# Autodesk Inventor assembly: #Spindexer
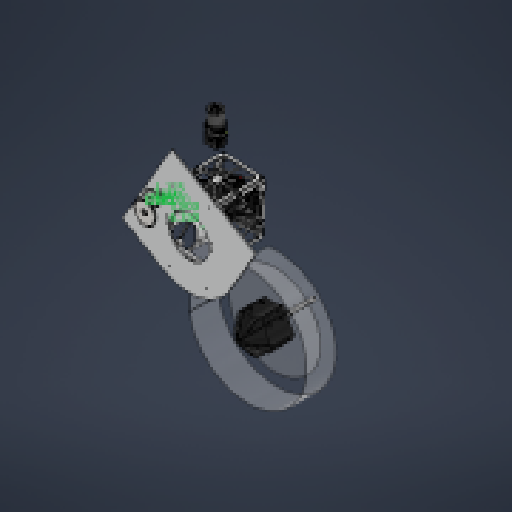
[picture p0: Inventor's stored thumbnail of the model, 512x512]
Saved by Autodesk Inventor 2026 (Build 300175000, 175)
## iProperties
Created: 2026-02-05
Part Number: #Spindexer
Document SubType Name: Assembly
Designer: Owen L
Mass: 5238.72 g
Surface Area: 14057.1 cm^2
Volume: 4457.84 cm^3
Density: 1.17517 g/cm^3
Author: Owen L
## Documents named in this file (44)
- C:\Users\littl\OneDrive\Documents\GitHub\2026-Robot-Mechanical\Spindexer\#Spindexer.iam
- C:\Users\littl\OneDrive\Documents\GitHub\2026-Robot-Mechanical\Spindexer\3DPRINT,HUB.ipt
- C:\Users\littl\OneDrive\Documents\GitHub\2026-Robot-Mechanical\Spindexer\3DPRINT,HUB,CONE.ipt
- C:\Users\littl\OneDrive\Documents\GitHub\2026-Robot-Mechanical\Spindexer\PLATE,WALL.ipt
- C:\Users\littl\OneDrive\Documents\GitHub\2026-Robot-Mechanical\Spindexer\PLATE,BOTTOM.ipt
- C:\Users\littl\OneDrive\Documents\GitHub\2026-Robot-Mechanical\Spindexer\STOCK,HEX,SHAFT,HUB.ipt
- C:\Users\littl\OneDrive\Documents\GitHub\2026-Robot-Mechanical\Spindexer\TEMP,BASE-SKETCH,TANGENT-OUT.ipt
- C:\Users\littl\OneDrive\Documents\GitHub\2026-Robot-Mechanical\Spindexer\PLATE,KICKER,OUTSIDE.ipt
- C:\Users\littl\OneDrive\Documents\GitHub\2026-Robot-Mechanical\Spindexer\3DPRINT,KICKER,RAMP.ipt
- C:\Users\littl\OneDrive\Documents\GitHub\2026-Robot-Mechanical\Spindexer\PLATE,KICKER,INSIDE.ipt
- C:\Users\littl\OneDrive\Documents\GitHub\2026-Robot-Mechanical\Spindexer\STOCK,HEX,SHAFT,KICKER,FRONT.ipt
- C:\Users\littl\OneDrive\Documents\GitHub\2026-Robot-Mechanical\Spindexer\STOCK,HEX,SHAFT,KICKER,BACK.ipt
- C:\Users\littl\OneDrive\Documents\GitHub\2026-Robot-Mechanical\#1_CAD Library\Power Transmission\Bearings\PURCHASED,HEX_BEARING.ipt
- C:\Users\littl\OneDrive\Documents\GitHub\2026-Robot-Mechanical\#1_CAD Library\Power Transmission\VersaPlanetary\GEARBOX,VERSAPLANETARY,SINGLE-STAGE,HEX-SHAFT,0.5IN.ipt
- C:\Users\littl\OneDrive\Documents\GitHub\2026-Robot-Mechanical\#1_CAD Library\Power Transmission\VersaPlanetary\ADAPTER,CIM-NEO,VERSAPLANETARY.ipt
- C:\Users\littl\OneDrive\Documents\GitHub\2026-Robot-Mechanical\#1_CAD Library\Motors\MOTOR,REV,NEO,V1-1.ipt
- C:\Users\littl\OneDrive\Documents\GitHub\2026-Robot-Mechanical\Spindexer\PLATE,NUT-BLOCK,3-LONG.ipt
- C:\Users\littl\OneDrive\Documents\GitHub\2026-Robot-Mechanical\Spindexer\PLATE,NUT-BLOCK,2-LONG.ipt
- C:\Users\littl\OneDrive\Documents\GitHub\2026-Robot-Mechanical\Spindexer\PLATE,NUT-BLOCK,1-LONG.ipt
- C:\Users\littl\OneDrive\Documents\GitHub\2026-Robot-Mechanical\#1_CAD Library\Electronics\CONTROLS,SPARK_MAX.ipt
- C:\Users\littl\OneDrive\Documents\GitHub\2026-Robot-Mechanical\Spindexer\3DPRINT,SPARK_MAX,MOUNT.ipt
- C:\Users\littl\OneDrive\Documents\GitHub\2026-Robot-Mechanical\Spindexer\PLATE,KICKER,BACK.ipt
- C:\Users\littl\OneDrive\Documents\GitHub\2026-Robot-Mechanical\Spindexer\PLATE,NUT-BLOCK,L-SHAPE.ipt
- C:\Users\littl\OneDrive\Documents\GitHub\2026-Robot-Mechanical\Spindexer\3DPRINTED,PULLEY,21T,9mm.ipt
- C:\Users\littl\OneDrive\Documents\GitHub\2026-Robot-Mechanical\#1_CAD Library\Power Transmission\Pulleys\PURCHASED,HTD5mm,24T,PULLEY.ipt
- C:\Users\littl\OneDrive\Documents\GitHub\2026-Robot-Mechanical\Spindexer\STANDIN,BELT,70T,HTD5mm.ipt
- C:\Users\littl\OneDrive\Documents\GitHub\2026-Robot-Mechanical\Spindexer\STANDIN,BELT,100T,HTD5mm.ipt
- C:\Users\littl\OneDrive\Documents\GitHub\2026-Robot-Mechanical\#1_CAD Library\Building Materials\Fasteners\Bolts\PURCHASED,10-32x0.5in,BUTTONHEAD,BOLT.ipt
- C:\Users\littl\OneDrive\Documents\GitHub\2026-Robot-Mechanical\#1_CAD Library\Building Materials\Fasteners\Nuts\PURCHASED,NYLOCK,10-32,NUT.ipt
- C:\Users\littl\OneDrive\Documents\GitHub\2026-Robot-Mechanical\#1_CAD Library\Building Materials\Fasteners\Bolts\PURCHASED,10-32x0.625in,BUTTONHEAD,BOLT.ipt
- C:\Users\littl\OneDrive\Documents\GitHub\2026-Robot-Mechanical\Spindexer\PLATE,NUT-BLOCK,SINGLE-L.ipt
- C:\Users\littl\OneDrive\Documents\GitHub\2026-Robot-Mechanical\Spindexer\PLATE,SHOOTER,MOUNT.ipt
- C:\Users\littl\OneDrive\Documents\GitHub\2026-Robot-Mechanical\Spindexer\#Spindexer\Design Accelerator\PLATE,TURRET,ENCODER,GEAR.ipt
- C:\Users\littl\OneDrive\Documents\GitHub\2026-Robot-Mechanical\Spindexer\#Spindexer\Design Accelerator\PLATE,TURRET,PINNION,GEAR.ipt
- C:\Users\littl\OneDrive\Documents\GitHub\2026-Robot-Mechanical\Spindexer\#Spindexer\Design Accelerator\PLATE,TURRET,MOTOR,MOUNT.ipt
- C:\Users\littl\OneDrive\Documents\GitHub\2026-Robot-Mechanical\#1_CAD Library\Electronics\CONTROLS,ENCODER,HEX_BORE.ipt
- C:\Users\littl\OneDrive\Documents\GitHub\2026-Robot-Mechanical\Spindexer\#Spindexer\Design Accelerator\STOCK,HEX,SHAFT,TURRET,DRIVE.ipt
- C:\Users\littl\OneDrive\Documents\GitHub\2026-Robot-Mechanical\Spindexer\#Spindexer\Design Accelerator\STOCK,HEX,SHAFT,TURRET,ENCODER.ipt
- C:\Users\littl\OneDrive\Documents\GitHub\2026-Robot-Mechanical\Spindexer\#Spindexer\Design Accelerator\3DPRINT,TURRET,HEX,SPACER.ipt
- C:\Users\littl\OneDrive\Documents\GitHub\2026-Robot-Mechanical\Spindexer\MOTOR,NEO,VORTEX,WITH-MAX-PLANETARY.ipt
- C:\Users\littl\OneDrive\Documents\GitHub\2026-Robot-Mechanical\Spindexer\STOCK,CHURRO,HEX,TURRET,MOTOR-MOUNT,SPACER.ipt
- C:\Users\littl\OneDrive\Documents\GitHub\2026-Robot-Mechanical\#1_CAD Library\Building Materials\Fasteners\Bolts\PURCHASED,0.25-20x0.5in,BUTTONHEAD,BOLT.ipt
- C:\Users\littl\OneDrive\Documents\GitHub\2026-Robot-Mechanical\Spindexer\3DRPINT,FRONT-ROLLER,DRIVE-SPACER.ipt
- C:\Users\littl\OneDrive\Documents\GitHub\2026-Robot-Mechanical\Spindexer\CAST,SLAB-OF-FLOP.ipt
## Components (132 placed, 43 different names)
1. 3DPRINT,HUB:1 — Mate:11, Mate:12, Mate:13, Mate:15, Mate:16, Mate:17, Flush:2, Mate:18, Mate:19, Mate:106, Mate:107, Mate:108, Mate:109, Mate:110, Mate:111, Mate:112, Mate:113, Mate:114, Mate:115
2. 3DPRINT,HUB,CONE:1 — Mate:11, Mate:12, Mate:13
3. PLATE,WALL:1 — Mate:32, Flush:7, Flush:8, Mate:42, Mate:43
4. PLATE,BOTTOM:1 — Mate:18, Mate:19, Mate:32, Flush:7
5. STOCK,HEX,SHAFT,HUB:1 — Mate:16, Mate:17, Flush:2
6. TEMP,BASE-SKETCH,TANGENT-OUT:1
7. PLATE,KICKER,OUTSIDE:1 — Mate:22, Mate:23, Mate:24, Mate:25, Flush:3, Flush:4, Flush:8, Insert:1, Insert:4, Mate:34, Mate:35, Mate:42, Insert:9, Insert:10, Insert:13, Flush:12, Mate:43, Insert:23, Insert:24, Insert:34, Insert:35, Insert:39, Insert:40, Insert:41, Insert:42, Insert:43, Insert:44, Insert:45, Insert:46, Insert:47, Insert:48, Insert:49, Insert:50, Insert:79, Insert:80, Insert:81, Insert:82, Mate:59, Insert:83, Mate:62, Insert:87, Insert:93, Insert:94, Insert:98, Insert:99, Insert:100, Mate:65
8. 3DPRINT,KICKER,RAMP:1 — Mate:22, Mate:23, Mate:24
9. PLATE,KICKER,INSIDE:1 — Mate:25, Flush:3, Flush:4, Insert:2, Insert:3, Mate:39, Mate:40, Mate:41, Insert:14, Insert:21, Insert:22, Insert:31, Insert:32, Insert:33, Mate:48, Mate:52, Insert:61, Insert:65, Insert:66, Insert:67, Insert:68, Insert:69, Insert:70, Insert:71, Insert:72, Insert:73, Insert:74, Insert:75, Insert:76, Insert:77, Insert:78, Mate:60, Insert:84, Mate:61, Insert:90, Insert:91, Insert:92, Insert:95, Insert:96, Insert:97
10. STOCK,HEX,SHAFT,KICKER,FRONT:1 — Mate:34, Mate:45, Flush:15
11. STOCK,HEX,SHAFT,KICKER,BACK:1 — Mate:35, Mate:46, Mate:47, Flush:14
12. PURCHASED,HEX_BEARING:1 — Insert:1, Flush:15
13. PURCHASED,HEX_BEARING:2 — Insert:2, Mate:103, Mate:104
14. PURCHASED,HEX_BEARING:3 — Insert:3, Mate:63
15. PURCHASED,HEX_BEARING:4 — Insert:4, Flush:14
16. GEARBOX,VERSAPLANETARY,SINGLE-STAGE,HEX-SHAFT,0.5IN:1 — Mate:36, Mate:37, Mate:38, Mate:39, Mate:40, Mate:41, Mate:53
17. ADAPTER,CIM-NEO,VERSAPLANETARY:1 — Mate:36, Mate:37, Mate:38, Insert:5
18. MOTOR,REV,NEO,V1-1:1 — Insert:5
19. PLATE,NUT-BLOCK,3-LONG:1 — Mate:60, Insert:84
20. PLATE,NUT-BLOCK,3-LONG:2 — Insert:9, Insert:10
21. PLATE,NUT-BLOCK,3-LONG:3 — Mate:59, Insert:83
22. PLATE,NUT-BLOCK,1-LONG:1 — Insert:13, Flush:11, Flush:12
23. PLATE,NUT-BLOCK,1-LONG:2 — Insert:14, Flush:11
24. PLATE,NUT-BLOCK,3-LONG:4 — Insert:91, Insert:92, Mate:66
25. PLATE,NUT-BLOCK,3-LONG:5 — Insert:93, Insert:94, Mate:67
26. CONTROLS,SPARK_MAX:1
27. 3DPRINT,SPARK_MAX,MOUNT:1
28. PLATE,KICKER,BACK:1 — Mate:44, Insert:25, Insert:26, Insert:27, Insert:28, Insert:51, Insert:52, Insert:53, Insert:54, Insert:55, Insert:59, Insert:60, Insert:85, Insert:86, Insert:88, Insert:89
29. PLATE,NUT-BLOCK,2-LONG:2 — Insert:21, Insert:22, Mate:44, Insert:26
30. PLATE,NUT-BLOCK,2-LONG:3 — Insert:23, Insert:24, Insert:25
31. PLATE,NUT-BLOCK,3-LONG:6 — Insert:27, Insert:28
32. PLATE,NUT-BLOCK,3-LONG:8 — Insert:31, Insert:32
33. PLATE,NUT-BLOCK,L-SHAPE:1 — Insert:33
34. PLATE,NUT-BLOCK,L-SHAPE:2 — Insert:34
35. 3DPRINTED,PULLEY,21T,9mm:1 — Mate:46, Mate:55, Mate:58, Mate:64, Flush:16
36. 3DPRINTED,PULLEY,21T,9mm:2 — Mate:45, Mate:54, Flush:16
37. PURCHASED,HEX_BEARING:5 — Mate:52, Mate:53
38. PURCHASED,HTD5mm,24T,PULLEY:1 — Mate:47, Flush:13, Mate:57, Mate:63, Mate:64
39. PURCHASED,HTD5mm,24T,PULLEY:2 — Mate:48, Flush:13, Mate:56
40. STANDIN,BELT,70T,HTD5mm:1 — Mate:56, Mate:57
41. STANDIN,BELT,100T,HTD5mm:1 — Mate:54, Mate:55, Mate:58
42. PURCHASED,10-32x0.5in,BUTTONHEAD,BOLT:1 — Insert:48
43. PURCHASED,NYLOCK,10-32,NUT:1 — Insert:81
44. PURCHASED,10-32x0.625in,BUTTONHEAD,BOLT:1 — Insert:35
45. PURCHASED,10-32x0.625in,BUTTONHEAD,BOLT:5 — Insert:39
46. PURCHASED,10-32x0.625in,BUTTONHEAD,BOLT:6 — Insert:40
47. PURCHASED,10-32x0.625in,BUTTONHEAD,BOLT:7 — Insert:41
48. PURCHASED,10-32x0.625in,BUTTONHEAD,BOLT:8 — Insert:42
49. PURCHASED,10-32x0.625in,BUTTONHEAD,BOLT:9 — Insert:43
50. PURCHASED,10-32x0.625in,BUTTONHEAD,BOLT:10 — Insert:44
51. PURCHASED,10-32x0.625in,BUTTONHEAD,BOLT:11 — Insert:45
52. PURCHASED,10-32x0.625in,BUTTONHEAD,BOLT:12 — Insert:46
53. PURCHASED,10-32x0.625in,BUTTONHEAD,BOLT:13 — Insert:47
54. PURCHASED,10-32x0.625in,BUTTONHEAD,BOLT:14 — Insert:51
55. PURCHASED,10-32x0.625in,BUTTONHEAD,BOLT:15 — Insert:52
56. PURCHASED,10-32x0.625in,BUTTONHEAD,BOLT:16 — Insert:53
57. PURCHASED,10-32x0.625in,BUTTONHEAD,BOLT:17 — Insert:54
58. PURCHASED,10-32x0.625in,BUTTONHEAD,BOLT:18 — Insert:55
59. PURCHASED,10-32x0.5in,BUTTONHEAD,BOLT:2 — Insert:49
60. PURCHASED,10-32x0.5in,BUTTONHEAD,BOLT:3 — Insert:50
61. PURCHASED,10-32x0.625in,BUTTONHEAD,BOLT:19 — Insert:59
62. PURCHASED,10-32x0.625in,BUTTONHEAD,BOLT:20 — Insert:89
63. PURCHASED,10-32x0.625in,BUTTONHEAD,BOLT:21 — Insert:87
64. PURCHASED,10-32x0.625in,BUTTONHEAD,BOLT:22 — Insert:60
65. PURCHASED,10-32x0.625in,BUTTONHEAD,BOLT:23 — Insert:88
66. PURCHASED,10-32x0.625in,BUTTONHEAD,BOLT:24 — Insert:61
67. PURCHASED,10-32x0.625in,BUTTONHEAD,BOLT:28 — Insert:65
68. PURCHASED,10-32x0.625in,BUTTONHEAD,BOLT:29 — Insert:66
69. PURCHASED,10-32x0.625in,BUTTONHEAD,BOLT:30 — Insert:67
70. PURCHASED,10-32x0.625in,BUTTONHEAD,BOLT:31 — Insert:68
71. PURCHASED,10-32x0.625in,BUTTONHEAD,BOLT:32 — Insert:69
72. PURCHASED,10-32x0.625in,BUTTONHEAD,BOLT:33 — Insert:70
73. PURCHASED,10-32x0.625in,BUTTONHEAD,BOLT:34 — Insert:73
74. PURCHASED,10-32x0.625in,BUTTONHEAD,BOLT:35 — Insert:72
75. PURCHASED,10-32x0.625in,BUTTONHEAD,BOLT:36 — Insert:71
76. PURCHASED,10-32x0.5in,BUTTONHEAD,BOLT:4 — Insert:74
77. PURCHASED,10-32x0.5in,BUTTONHEAD,BOLT:5 — Insert:76
78. PURCHASED,10-32x0.5in,BUTTONHEAD,BOLT:6 — Insert:75
79. PURCHASED,10-32x0.5in,BUTTONHEAD,BOLT:7 — Insert:77
80. PURCHASED,10-32x0.5in,BUTTONHEAD,BOLT:8 — Insert:78
81. PURCHASED,10-32x0.5in,BUTTONHEAD,BOLT:9 — Insert:79
82. PURCHASED,10-32x0.5in,BUTTONHEAD,BOLT:10 — Insert:80
83. PURCHASED,NYLOCK,10-32,NUT:2 — Insert:82
84. PLATE,NUT-BLOCK,SINGLE-L:1 — Insert:85, Mate:61
85. PLATE,NUT-BLOCK,SINGLE-L:2 — Insert:86, Mate:62
86. PURCHASED,10-32x0.625in,BUTTONHEAD,BOLT:37 — Insert:90
87. PURCHASED,10-32x0.625in,BUTTONHEAD,BOLT:38 — Insert:95
88. PURCHASED,10-32x0.625in,BUTTONHEAD,BOLT:39 — Insert:96
89. PURCHASED,10-32x0.625in,BUTTONHEAD,BOLT:40 — Insert:97
90. PURCHASED,10-32x0.625in,BUTTONHEAD,BOLT:41 — Insert:98
91. PURCHASED,10-32x0.625in,BUTTONHEAD,BOLT:42 — Insert:99
92. PURCHASED,10-32x0.625in,BUTTONHEAD,BOLT:43 — Insert:100
93. PLATE,SHOOTER,MOUNT:1 — Mate:65, Mate:66, Mate:67, Insert:101, Insert:102, Mate:82, Mate:85, Insert:118, Insert:119, Mate:95, Mate:97, Mate:98, Mate:99, Mate:100, Insert:122, Insert:123, Insert:124, Insert:125, Insert:126, Insert:128, Insert:129, Insert:130, Mate:105, Insert:136, Insert:137
94. PLATE,TURRET,ENCODER,GEAR:1 — Mate:85, Flush:20, Mate:89, Mate:102
95. PLATE,TURRET,PINNION,GEAR:1 — Mate:86, Flush:18, Mate:88
96. PURCHASED,HEX_BEARING:6 — Insert:101, Mate:83, Mate:86, Mate:93
97. PURCHASED,HEX_BEARING:7 — Insert:102, Mate:94, Mate:96
98. PLATE,TURRET,MOTOR,MOUNT:1 — Mate:98, Mate:99, Insert:120, Mate:100, Insert:121, Mate:101, Insert:127, Insert:131, Insert:132, Insert:133
99. CONTROLS,ENCODER,HEX_BORE:1 — Mate:95, Mate:96, Mate:97, Insert:135, Insert:134
100. CONTROLS,ENCODER,HEX_BORE:2 — Mate:82, Mate:83, Mate:87, Insert:112, Insert:113
101. STOCK,HEX,SHAFT,TURRET,DRIVE:1 — Flush:20, Mate:89, Mate:91
102. STOCK,HEX,SHAFT,TURRET,ENCODER:1 — Flush:18, Mate:87, Mate:88, Mate:92, Flush:21
103. 3DPRINT,TURRET,HEX,SPACER:1 — Mate:91, Mate:94, Mate:102
104. 3DPRINT,TURRET,HEX,SPACER:2 — Mate:92, Mate:93
105. PURCHASED,10-32x0.625in,BUTTONHEAD,BOLT:44 — Insert:112, Mate:105
106. PURCHASED,10-32x0.625in,BUTTONHEAD,BOLT:45 — Insert:113
107. PURCHASED,NYLOCK,10-32,NUT:5 — Insert:118
108. PURCHASED,NYLOCK,10-32,NUT:6 — Insert:119
109. MOTOR,NEO,VORTEX,WITH-MAX-PLANETARY:1 — Insert:121, Mate:101
110. PURCHASED,HEX_BEARING:9 — Insert:120, Flush:21
111. STOCK,CHURRO,HEX,TURRET,MOTOR-MOUNT,SPACER:1 — Insert:122
112. STOCK,CHURRO,HEX,TURRET,MOTOR-MOUNT,SPACER:2 — Insert:123
113. STOCK,CHURRO,HEX,TURRET,MOTOR-MOUNT,SPACER:3 — Insert:124
114. STOCK,CHURRO,HEX,TURRET,MOTOR-MOUNT,SPACER:4 — Insert:125
115. PURCHASED,0.25-20x0.5in,BUTTONHEAD,BOLT:1 — Insert:132
116. PURCHASED,0.25-20x0.5in,BUTTONHEAD,BOLT:2 — Insert:133
117. PURCHASED,0.25-20x0.5in,BUTTONHEAD,BOLT:3 — Insert:131
118. PURCHASED,0.25-20x0.5in,BUTTONHEAD,BOLT:4 — Insert:130
119. PURCHASED,0.25-20x0.5in,BUTTONHEAD,BOLT:5 — Insert:129
120. PURCHASED,0.25-20x0.5in,BUTTONHEAD,BOLT:6 — Insert:128
121. PURCHASED,0.25-20x0.5in,BUTTONHEAD,BOLT:7 — Insert:127
122. PURCHASED,0.25-20x0.5in,BUTTONHEAD,BOLT:8 — Insert:126
123. 3DRPINT,FRONT-ROLLER,DRIVE-SPACER:1 — Mate:103, Mate:104
124. PURCHASED,10-32x0.625in,BUTTONHEAD,BOLT:46 — Insert:134
125. PURCHASED,10-32x0.625in,BUTTONHEAD,BOLT:47 — Insert:135
126. PURCHASED,NYLOCK,10-32,NUT:7 — Insert:136
127. PURCHASED,NYLOCK,10-32,NUT:8 — Insert:137
128. CAST,SLAB-OF-FLOP:1 — Mate:106, Mate:107
129. CAST,SLAB-OF-FLOP:2 — Mate:108, Mate:109
130. CAST,SLAB-OF-FLOP:3 — Mate:110, Mate:111
131. CAST,SLAB-OF-FLOP:4 — Mate:112, Mate:113
132. CAST,SLAB-OF-FLOP:5 — Mate:114, Mate:115
## Relationships (192: Insert 102, Mate 76, Flush 14)
- Mate:11: 3DPRINT,HUB:1 ↔ 3DPRINT,HUB,CONE:1
- Mate:12: 3DPRINT,HUB:1 ↔ 3DPRINT,HUB,CONE:1
- Mate:13: 3DPRINT,HUB:1 ↔ 3DPRINT,HUB,CONE:1
- Mate:15: 3DPRINT,HUB:1
- Mate:16: 3DPRINT,HUB:1 ↔ STOCK,HEX,SHAFT,HUB:1
- Mate:17: 3DPRINT,HUB:1 ↔ STOCK,HEX,SHAFT,HUB:1
- Flush:2 (-12.7 mm): 3DPRINT,HUB:1 ↔ STOCK,HEX,SHAFT,HUB:1
- Mate:18: 3DPRINT,HUB:1 ↔ PLATE,BOTTOM:1
- Mate:19: 3DPRINT,HUB:1 ↔ PLATE,BOTTOM:1
- Mate:22: PLATE,KICKER,OUTSIDE:1 ↔ 3DPRINT,KICKER,RAMP:1
- Mate:23: PLATE,KICKER,OUTSIDE:1 ↔ 3DPRINT,KICKER,RAMP:1
- Mate:24: PLATE,KICKER,OUTSIDE:1 ↔ 3DPRINT,KICKER,RAMP:1
- Mate:25 (158.75 mm): PLATE,KICKER,OUTSIDE:1 ↔ PLATE,KICKER,INSIDE:1
- Flush:3: PLATE,KICKER,OUTSIDE:1 ↔ PLATE,KICKER,INSIDE:1
- Flush:4: PLATE,KICKER,OUTSIDE:1 ↔ PLATE,KICKER,INSIDE:1
- Mate:32: PLATE,WALL:1 ↔ PLATE,BOTTOM:1
- Flush:7 (-6.35 mm): PLATE,WALL:1 ↔ PLATE,BOTTOM:1
- Flush:8: PLATE,WALL:1 ↔ PLATE,KICKER,OUTSIDE:1
- Insert:1: PLATE,KICKER,OUTSIDE:1 ↔ PURCHASED,HEX_BEARING:1
- Insert:2: PLATE,KICKER,INSIDE:1 ↔ PURCHASED,HEX_BEARING:2
- Insert:3: PLATE,KICKER,INSIDE:1 ↔ PURCHASED,HEX_BEARING:3
- Insert:4: PLATE,KICKER,OUTSIDE:1 ↔ PURCHASED,HEX_BEARING:4
- Mate:34: PLATE,KICKER,OUTSIDE:1 ↔ STOCK,HEX,SHAFT,KICKER,FRONT:1
- Mate:35: PLATE,KICKER,OUTSIDE:1 ↔ STOCK,HEX,SHAFT,KICKER,BACK:1
- Mate:36: GEARBOX,VERSAPLANETARY,SINGLE-STAGE,HEX-SHAFT,0.5IN:1 ↔ ADAPTER,CIM-NEO,VERSAPLANETARY:1
- Mate:37: GEARBOX,VERSAPLANETARY,SINGLE-STAGE,HEX-SHAFT,0.5IN:1 ↔ ADAPTER,CIM-NEO,VERSAPLANETARY:1
- Mate:38: GEARBOX,VERSAPLANETARY,SINGLE-STAGE,HEX-SHAFT,0.5IN:1 ↔ ADAPTER,CIM-NEO,VERSAPLANETARY:1
- Insert:5: ADAPTER,CIM-NEO,VERSAPLANETARY:1 ↔ MOTOR,REV,NEO,V1-1:1
- Mate:39: PLATE,KICKER,INSIDE:1 ↔ GEARBOX,VERSAPLANETARY,SINGLE-STAGE,HEX-SHAFT,0.5IN:1
- Mate:40: PLATE,KICKER,INSIDE:1 ↔ GEARBOX,VERSAPLANETARY,SINGLE-STAGE,HEX-SHAFT,0.5IN:1
- Mate:41: PLATE,KICKER,INSIDE:1 ↔ GEARBOX,VERSAPLANETARY,SINGLE-STAGE,HEX-SHAFT,0.5IN:1
- Mate:42: PLATE,WALL:1 ↔ PLATE,KICKER,OUTSIDE:1
- Insert:9: PLATE,KICKER,OUTSIDE:1 ↔ PLATE,NUT-BLOCK,3-LONG:2
- Insert:10: PLATE,KICKER,OUTSIDE:1 ↔ PLATE,NUT-BLOCK,3-LONG:2
- Insert:13: PLATE,KICKER,OUTSIDE:1 ↔ PLATE,NUT-BLOCK,1-LONG:1
- Insert:14: PLATE,KICKER,INSIDE:1 ↔ PLATE,NUT-BLOCK,1-LONG:2
- Flush:11: PLATE,NUT-BLOCK,1-LONG:1 ↔ PLATE,NUT-BLOCK,1-LONG:2
- Flush:12: PLATE,KICKER,OUTSIDE:1 ↔ PLATE,NUT-BLOCK,1-LONG:1
- Mate:43 (-25.4 mm): PLATE,WALL:1 ↔ PLATE,KICKER,OUTSIDE:1
- Insert:21: PLATE,KICKER,INSIDE:1 ↔ PLATE,NUT-BLOCK,2-LONG:2
- Insert:22: PLATE,KICKER,INSIDE:1 ↔ PLATE,NUT-BLOCK,2-LONG:2
- Insert:23: PLATE,KICKER,OUTSIDE:1 ↔ PLATE,NUT-BLOCK,2-LONG:3
- Insert:24: PLATE,KICKER,OUTSIDE:1 ↔ PLATE,NUT-BLOCK,2-LONG:3
- Mate:44: PLATE,KICKER,BACK:1 ↔ PLATE,NUT-BLOCK,2-LONG:2
- Insert:25: PLATE,KICKER,BACK:1 ↔ PLATE,NUT-BLOCK,2-LONG:3
- Insert:26: PLATE,KICKER,BACK:1 ↔ PLATE,NUT-BLOCK,2-LONG:2
- Insert:27: PLATE,KICKER,BACK:1 ↔ PLATE,NUT-BLOCK,3-LONG:6
- Insert:28: PLATE,KICKER,BACK:1 ↔ PLATE,NUT-BLOCK,3-LONG:6
- Insert:31: PLATE,KICKER,INSIDE:1 ↔ PLATE,NUT-BLOCK,3-LONG:8
- Insert:32: PLATE,KICKER,INSIDE:1 ↔ PLATE,NUT-BLOCK,3-LONG:8
- Insert:33: PLATE,KICKER,INSIDE:1 ↔ PLATE,NUT-BLOCK,L-SHAPE:1
- Insert:34: PLATE,KICKER,OUTSIDE:1 ↔ PLATE,NUT-BLOCK,L-SHAPE:2
- Mate:45: STOCK,HEX,SHAFT,KICKER,FRONT:1 ↔ 3DPRINTED,PULLEY,21T,9mm:2
- Mate:46: STOCK,HEX,SHAFT,KICKER,BACK:1 ↔ 3DPRINTED,PULLEY,21T,9mm:1
- Mate:47: STOCK,HEX,SHAFT,KICKER,BACK:1 ↔ PURCHASED,HTD5mm,24T,PULLEY:1
- Mate:48: PLATE,KICKER,INSIDE:1 ↔ PURCHASED,HTD5mm,24T,PULLEY:2
- Flush:13: PURCHASED,HTD5mm,24T,PULLEY:1 ↔ PURCHASED,HTD5mm,24T,PULLEY:2
- Flush:14: STOCK,HEX,SHAFT,KICKER,BACK:1 ↔ PURCHASED,HEX_BEARING:4
- Flush:15: STOCK,HEX,SHAFT,KICKER,FRONT:1 ↔ PURCHASED,HEX_BEARING:1
- Mate:52: PLATE,KICKER,INSIDE:1 ↔ PURCHASED,HEX_BEARING:5
- Mate:53: GEARBOX,VERSAPLANETARY,SINGLE-STAGE,HEX-SHAFT,0.5IN:1 ↔ PURCHASED,HEX_BEARING:5
- Mate:54: 3DPRINTED,PULLEY,21T,9mm:2 ↔ STANDIN,BELT,100T,HTD5mm:1
- Mate:55: 3DPRINTED,PULLEY,21T,9mm:1 ↔ STANDIN,BELT,100T,HTD5mm:1
- Mate:56: PURCHASED,HTD5mm,24T,PULLEY:2 ↔ STANDIN,BELT,70T,HTD5mm:1
- Mate:57: PURCHASED,HTD5mm,24T,PULLEY:1 ↔ STANDIN,BELT,70T,HTD5mm:1
- Mate:58: 3DPRINTED,PULLEY,21T,9mm:1 ↔ STANDIN,BELT,100T,HTD5mm:1
- Insert:35: PLATE,KICKER,OUTSIDE:1 ↔ PURCHASED,10-32x0.625in,BUTTONHEAD,BOLT:1
- Insert:39: PLATE,KICKER,OUTSIDE:1 ↔ PURCHASED,10-32x0.625in,BUTTONHEAD,BOLT:5
- Insert:40: PLATE,KICKER,OUTSIDE:1 ↔ PURCHASED,10-32x0.625in,BUTTONHEAD,BOLT:6
- Insert:41: PLATE,KICKER,OUTSIDE:1 ↔ PURCHASED,10-32x0.625in,BUTTONHEAD,BOLT:7
- Insert:42: PLATE,KICKER,OUTSIDE:1 ↔ PURCHASED,10-32x0.625in,BUTTONHEAD,BOLT:8
- Insert:43: PLATE,KICKER,OUTSIDE:1 ↔ PURCHASED,10-32x0.625in,BUTTONHEAD,BOLT:9
- Insert:44: PLATE,KICKER,OUTSIDE:1 ↔ PURCHASED,10-32x0.625in,BUTTONHEAD,BOLT:10
- Insert:45: PLATE,KICKER,OUTSIDE:1 ↔ PURCHASED,10-32x0.625in,BUTTONHEAD,BOLT:11
- Insert:46: PLATE,KICKER,OUTSIDE:1 ↔ PURCHASED,10-32x0.625in,BUTTONHEAD,BOLT:12
- Insert:47: PLATE,KICKER,OUTSIDE:1 ↔ PURCHASED,10-32x0.625in,BUTTONHEAD,BOLT:13
- Insert:48: PLATE,KICKER,OUTSIDE:1 ↔ PURCHASED,10-32x0.5in,BUTTONHEAD,BOLT:1
- Insert:49: PLATE,KICKER,OUTSIDE:1 ↔ PURCHASED,10-32x0.5in,BUTTONHEAD,BOLT:2
- Insert:50: PLATE,KICKER,OUTSIDE:1 ↔ PURCHASED,10-32x0.5in,BUTTONHEAD,BOLT:3
- Insert:51: PLATE,KICKER,BACK:1 ↔ PURCHASED,10-32x0.625in,BUTTONHEAD,BOLT:14
- Insert:52: PLATE,KICKER,BACK:1 ↔ PURCHASED,10-32x0.625in,BUTTONHEAD,BOLT:15
- Insert:53: PLATE,KICKER,BACK:1 ↔ PURCHASED,10-32x0.625in,BUTTONHEAD,BOLT:16
- Insert:54: PLATE,KICKER,BACK:1 ↔ PURCHASED,10-32x0.625in,BUTTONHEAD,BOLT:17
- Insert:55: PLATE,KICKER,BACK:1 ↔ PURCHASED,10-32x0.625in,BUTTONHEAD,BOLT:18
- Insert:59: PLATE,KICKER,BACK:1 ↔ PURCHASED,10-32x0.625in,BUTTONHEAD,BOLT:19
- Insert:60: PLATE,KICKER,BACK:1 ↔ PURCHASED,10-32x0.625in,BUTTONHEAD,BOLT:22
- Insert:61: PLATE,KICKER,INSIDE:1 ↔ PURCHASED,10-32x0.625in,BUTTONHEAD,BOLT:24
- Insert:65: PLATE,KICKER,INSIDE:1 ↔ PURCHASED,10-32x0.625in,BUTTONHEAD,BOLT:28
- Insert:66: PLATE,KICKER,INSIDE:1 ↔ PURCHASED,10-32x0.625in,BUTTONHEAD,BOLT:29
- Insert:67: PLATE,KICKER,INSIDE:1 ↔ PURCHASED,10-32x0.625in,BUTTONHEAD,BOLT:30
- Insert:68: PLATE,KICKER,INSIDE:1 ↔ PURCHASED,10-32x0.625in,BUTTONHEAD,BOLT:31
- Insert:69: PLATE,KICKER,INSIDE:1 ↔ PURCHASED,10-32x0.625in,BUTTONHEAD,BOLT:32
- Insert:70: PLATE,KICKER,INSIDE:1 ↔ PURCHASED,10-32x0.625in,BUTTONHEAD,BOLT:33
- Insert:71: PLATE,KICKER,INSIDE:1 ↔ PURCHASED,10-32x0.625in,BUTTONHEAD,BOLT:36
- Insert:72: PLATE,KICKER,INSIDE:1 ↔ PURCHASED,10-32x0.625in,BUTTONHEAD,BOLT:35
- Insert:73: PLATE,KICKER,INSIDE:1 ↔ PURCHASED,10-32x0.625in,BUTTONHEAD,BOLT:34
- Insert:74: PLATE,KICKER,INSIDE:1 ↔ PURCHASED,10-32x0.5in,BUTTONHEAD,BOLT:4
- Insert:75: PLATE,KICKER,INSIDE:1 ↔ PURCHASED,10-32x0.5in,BUTTONHEAD,BOLT:6
- Insert:76: PLATE,KICKER,INSIDE:1 ↔ PURCHASED,10-32x0.5in,BUTTONHEAD,BOLT:5
- Insert:77: PLATE,KICKER,INSIDE:1 ↔ PURCHASED,10-32x0.5in,BUTTONHEAD,BOLT:7
- Insert:78: PLATE,KICKER,INSIDE:1 ↔ PURCHASED,10-32x0.5in,BUTTONHEAD,BOLT:8
- Insert:79: PLATE,KICKER,OUTSIDE:1 ↔ PURCHASED,10-32x0.5in,BUTTONHEAD,BOLT:9
- Insert:80: PLATE,KICKER,OUTSIDE:1 ↔ PURCHASED,10-32x0.5in,BUTTONHEAD,BOLT:10
- Insert:81: PLATE,KICKER,OUTSIDE:1 ↔ PURCHASED,NYLOCK,10-32,NUT:1
- Insert:82: PLATE,KICKER,OUTSIDE:1 ↔ PURCHASED,NYLOCK,10-32,NUT:2
- Mate:59: PLATE,KICKER,OUTSIDE:1 ↔ PLATE,NUT-BLOCK,3-LONG:3
- Insert:83: PLATE,KICKER,OUTSIDE:1 ↔ PLATE,NUT-BLOCK,3-LONG:3
- Mate:60: PLATE,KICKER,INSIDE:1 ↔ PLATE,NUT-BLOCK,3-LONG:1
- Insert:84: PLATE,KICKER,INSIDE:1 ↔ PLATE,NUT-BLOCK,3-LONG:1
- Insert:85: PLATE,KICKER,BACK:1 ↔ PLATE,NUT-BLOCK,SINGLE-L:1
- Mate:61: PLATE,KICKER,INSIDE:1 ↔ PLATE,NUT-BLOCK,SINGLE-L:1
- Insert:86: PLATE,KICKER,BACK:1 ↔ PLATE,NUT-BLOCK,SINGLE-L:2
- Mate:62: PLATE,KICKER,OUTSIDE:1 ↔ PLATE,NUT-BLOCK,SINGLE-L:2
- Insert:87: PLATE,KICKER,OUTSIDE:1 ↔ PURCHASED,10-32x0.625in,BUTTONHEAD,BOLT:21
- Insert:88: PLATE,KICKER,BACK:1 ↔ PURCHASED,10-32x0.625in,BUTTONHEAD,BOLT:23
- Insert:89: PLATE,KICKER,BACK:1 ↔ PURCHASED,10-32x0.625in,BUTTONHEAD,BOLT:20
- Insert:90: PLATE,KICKER,INSIDE:1 ↔ PURCHASED,10-32x0.625in,BUTTONHEAD,BOLT:37
- Mate:63: PURCHASED,HEX_BEARING:3 ↔ PURCHASED,HTD5mm,24T,PULLEY:1
- Mate:64: 3DPRINTED,PULLEY,21T,9mm:1 ↔ PURCHASED,HTD5mm,24T,PULLEY:1
- Flush:16: 3DPRINTED,PULLEY,21T,9mm:1 ↔ 3DPRINTED,PULLEY,21T,9mm:2
- Insert:91: PLATE,KICKER,INSIDE:1 ↔ PLATE,NUT-BLOCK,3-LONG:4
- Insert:92: PLATE,KICKER,INSIDE:1 ↔ PLATE,NUT-BLOCK,3-LONG:4
- Insert:93: PLATE,KICKER,OUTSIDE:1 ↔ PLATE,NUT-BLOCK,3-LONG:5
- Insert:94: PLATE,KICKER,OUTSIDE:1 ↔ PLATE,NUT-BLOCK,3-LONG:5
- Insert:95: PLATE,KICKER,INSIDE:1 ↔ PURCHASED,10-32x0.625in,BUTTONHEAD,BOLT:38
- Insert:96: PLATE,KICKER,INSIDE:1 ↔ PURCHASED,10-32x0.625in,BUTTONHEAD,BOLT:39
- Insert:97: PLATE,KICKER,INSIDE:1 ↔ PURCHASED,10-32x0.625in,BUTTONHEAD,BOLT:40
- Insert:98: PLATE,KICKER,OUTSIDE:1 ↔ PURCHASED,10-32x0.625in,BUTTONHEAD,BOLT:41
- Insert:99: PLATE,KICKER,OUTSIDE:1 ↔ PURCHASED,10-32x0.625in,BUTTONHEAD,BOLT:42
- Insert:100: PLATE,KICKER,OUTSIDE:1 ↔ PURCHASED,10-32x0.625in,BUTTONHEAD,BOLT:43
- Mate:65: PLATE,KICKER,OUTSIDE:1 ↔ PLATE,SHOOTER,MOUNT:1
- Mate:66: PLATE,NUT-BLOCK,3-LONG:4 ↔ PLATE,SHOOTER,MOUNT:1
- Mate:67: PLATE,NUT-BLOCK,3-LONG:5 ↔ PLATE,SHOOTER,MOUNT:1
- Insert:101: PLATE,SHOOTER,MOUNT:1 ↔ PURCHASED,HEX_BEARING:6
- Insert:102: PLATE,SHOOTER,MOUNT:1 ↔ PURCHASED,HEX_BEARING:7
- Mate:82: PLATE,SHOOTER,MOUNT:1 ↔ CONTROLS,ENCODER,HEX_BORE:2
- Mate:83: PURCHASED,HEX_BEARING:6 ↔ CONTROLS,ENCODER,HEX_BORE:2
- Mate:85: PLATE,SHOOTER,MOUNT:1 ↔ PLATE,TURRET,ENCODER,GEAR:1
- Mate:86: PLATE,TURRET,PINNION,GEAR:1 ↔ PURCHASED,HEX_BEARING:6
- Flush:18: PLATE,TURRET,PINNION,GEAR:1 ↔ STOCK,HEX,SHAFT,TURRET,ENCODER:1
- Mate:87: CONTROLS,ENCODER,HEX_BORE:2 ↔ STOCK,HEX,SHAFT,TURRET,ENCODER:1
- Mate:88: PLATE,TURRET,PINNION,GEAR:1 ↔ STOCK,HEX,SHAFT,TURRET,ENCODER:1
- Flush:20: PLATE,TURRET,ENCODER,GEAR:1 ↔ STOCK,HEX,SHAFT,TURRET,DRIVE:1
- Mate:89: PLATE,TURRET,ENCODER,GEAR:1 ↔ STOCK,HEX,SHAFT,TURRET,DRIVE:1
- Mate:91: STOCK,HEX,SHAFT,TURRET,DRIVE:1 ↔ 3DPRINT,TURRET,HEX,SPACER:1
- Mate:92: STOCK,HEX,SHAFT,TURRET,ENCODER:1 ↔ 3DPRINT,TURRET,HEX,SPACER:2
- Mate:93: PURCHASED,HEX_BEARING:6 ↔ 3DPRINT,TURRET,HEX,SPACER:2
- Mate:94: PURCHASED,HEX_BEARING:7 ↔ 3DPRINT,TURRET,HEX,SPACER:1
- Insert:112: CONTROLS,ENCODER,HEX_BORE:2 ↔ PURCHASED,10-32x0.625in,BUTTONHEAD,BOLT:44
- Insert:113: CONTROLS,ENCODER,HEX_BORE:2 ↔ PURCHASED,10-32x0.625in,BUTTONHEAD,BOLT:45
- Insert:118: PLATE,SHOOTER,MOUNT:1 ↔ PURCHASED,NYLOCK,10-32,NUT:5
- Insert:119: PLATE,SHOOTER,MOUNT:1 ↔ PURCHASED,NYLOCK,10-32,NUT:6
- Mate:95: PLATE,SHOOTER,MOUNT:1 ↔ CONTROLS,ENCODER,HEX_BORE:1
- Mate:96: PURCHASED,HEX_BEARING:7 ↔ CONTROLS,ENCODER,HEX_BORE:1
- Mate:97: PLATE,SHOOTER,MOUNT:1 ↔ CONTROLS,ENCODER,HEX_BORE:1
- Mate:98: PLATE,SHOOTER,MOUNT:1 ↔ PLATE,TURRET,MOTOR,MOUNT:1
- Mate:99: PLATE,SHOOTER,MOUNT:1 ↔ PLATE,TURRET,MOTOR,MOUNT:1
- Insert:120: PLATE,TURRET,MOTOR,MOUNT:1 ↔ PURCHASED,HEX_BEARING:9
- Mate:100 (17.78 mm): PLATE,SHOOTER,MOUNT:1 ↔ PLATE,TURRET,MOTOR,MOUNT:1
- Insert:121: PLATE,TURRET,MOTOR,MOUNT:1 ↔ MOTOR,NEO,VORTEX,WITH-MAX-PLANETARY:1
- Mate:101: PLATE,TURRET,MOTOR,MOUNT:1 ↔ MOTOR,NEO,VORTEX,WITH-MAX-PLANETARY:1
- Flush:21: STOCK,HEX,SHAFT,TURRET,ENCODER:1 ↔ PURCHASED,HEX_BEARING:9
- Mate:102: PLATE,TURRET,ENCODER,GEAR:1 ↔ 3DPRINT,TURRET,HEX,SPACER:1
- Insert:122: PLATE,SHOOTER,MOUNT:1 ↔ STOCK,CHURRO,HEX,TURRET,MOTOR-MOUNT,SPACER:1
- Insert:123: PLATE,SHOOTER,MOUNT:1 ↔ STOCK,CHURRO,HEX,TURRET,MOTOR-MOUNT,SPACER:2
- Insert:124: PLATE,SHOOTER,MOUNT:1 ↔ STOCK,CHURRO,HEX,TURRET,MOTOR-MOUNT,SPACER:3
- Insert:125: PLATE,SHOOTER,MOUNT:1 ↔ STOCK,CHURRO,HEX,TURRET,MOTOR-MOUNT,SPACER:4
- Insert:126: PLATE,SHOOTER,MOUNT:1 ↔ PURCHASED,0.25-20x0.5in,BUTTONHEAD,BOLT:8
- Insert:127: PLATE,TURRET,MOTOR,MOUNT:1 ↔ PURCHASED,0.25-20x0.5in,BUTTONHEAD,BOLT:7
- Insert:128: PLATE,SHOOTER,MOUNT:1 ↔ PURCHASED,0.25-20x0.5in,BUTTONHEAD,BOLT:6
- Insert:129: PLATE,SHOOTER,MOUNT:1 ↔ PURCHASED,0.25-20x0.5in,BUTTONHEAD,BOLT:5
- Insert:130: PLATE,SHOOTER,MOUNT:1 ↔ PURCHASED,0.25-20x0.5in,BUTTONHEAD,BOLT:4
- Insert:131: PLATE,TURRET,MOTOR,MOUNT:1 ↔ PURCHASED,0.25-20x0.5in,BUTTONHEAD,BOLT:3
- Insert:132: PLATE,TURRET,MOTOR,MOUNT:1 ↔ PURCHASED,0.25-20x0.5in,BUTTONHEAD,BOLT:1
- Insert:133: PLATE,TURRET,MOTOR,MOUNT:1 ↔ PURCHASED,0.25-20x0.5in,BUTTONHEAD,BOLT:2
- Mate:103: PURCHASED,HEX_BEARING:2 ↔ 3DRPINT,FRONT-ROLLER,DRIVE-SPACER:1
- Mate:104: PURCHASED,HEX_BEARING:2 ↔ 3DRPINT,FRONT-ROLLER,DRIVE-SPACER:1
- Mate:105: PLATE,SHOOTER,MOUNT:1 ↔ PURCHASED,10-32x0.625in,BUTTONHEAD,BOLT:44
- Insert:134: CONTROLS,ENCODER,HEX_BORE:1 ↔ PURCHASED,10-32x0.625in,BUTTONHEAD,BOLT:46
- Insert:135: CONTROLS,ENCODER,HEX_BORE:1 ↔ PURCHASED,10-32x0.625in,BUTTONHEAD,BOLT:47
- Insert:136: PLATE,SHOOTER,MOUNT:1 ↔ PURCHASED,NYLOCK,10-32,NUT:7
- Insert:137: PLATE,SHOOTER,MOUNT:1 ↔ PURCHASED,NYLOCK,10-32,NUT:8
- Mate:106: 3DPRINT,HUB:1 ↔ CAST,SLAB-OF-FLOP:1
- Mate:107: 3DPRINT,HUB:1 ↔ CAST,SLAB-OF-FLOP:1
- Mate:108: 3DPRINT,HUB:1 ↔ CAST,SLAB-OF-FLOP:2
- Mate:109: 3DPRINT,HUB:1 ↔ CAST,SLAB-OF-FLOP:2
- Mate:110: 3DPRINT,HUB:1 ↔ CAST,SLAB-OF-FLOP:3
- Mate:111: 3DPRINT,HUB:1 ↔ CAST,SLAB-OF-FLOP:3
- Mate:112: 3DPRINT,HUB:1 ↔ CAST,SLAB-OF-FLOP:4
- Mate:113: 3DPRINT,HUB:1 ↔ CAST,SLAB-OF-FLOP:4
- Mate:114: 3DPRINT,HUB:1 ↔ CAST,SLAB-OF-FLOP:5
- Mate:115: 3DPRINT,HUB:1 ↔ CAST,SLAB-OF-FLOP:5
